# Autodesk Inventor assembly: estrutura 4
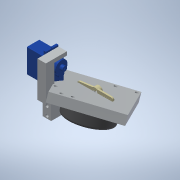
[picture p0: Inventor's stored thumbnail of the model, 180x180]
Saved by Autodesk Inventor 2021 (Build 250183000, 183)
## iProperties
Created: 2021-07-07
Part Number: estrutura 4
Document SubType Name: Assembly
Designer: Administrator
Title: estrutura 4
Author: Administrator
## Documents named in this file (6)
- C:\Users\ASUS\Desktop\base\estrutura 4.iam
- C:\Users\ASUS\Desktop\base\Arm 2.ipt
- C:\Users\ASUS\Desktop\base\Servomotor HTX900 - Cópia.ipt
- C:\Users\ASUS\Desktop\base\base da garra.ipt
- C:\Users\ASUS\Desktop\base\suporte do servo da garra.ipt
- C:\Users\ASUS\Desktop\robotic arm\Gripper v2.ipt
## Components (5 placed, 5 different names)
1. Arm 2:1 — Mate:1
2. Servomotor HTX900 - Cópia:3
3. base da garra:1 — Rotational:1, Mate:1
4. suporte do servo da garra:1
5. Gripper v2:1 — Rotational:1
## Relationships (2: RevoluteJoint 1, Mate 1)
- Rotational:1 [RevoluteJoint]: base da garra:1 ↔ Gripper v2:1
- Mate:1: Arm 2:1 ↔ base da garra:1
